# Autodesk Inventor assembly: dummy_pam_module_assembly
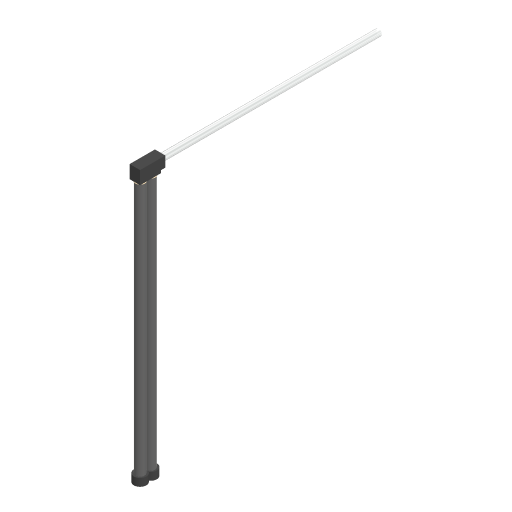
[picture p0: Inventor's stored thumbnail of the model, 512x512]
Saved by Autodesk Inventor 2024.3 (Build 283343000, 343)
## iProperties
Created: 2024-09-12
Part Number: dummy_pam_module_assembly
Document SubType Name: Assembly
Designer: gihyeok2
Author: gihyeok2
## Documents named in this file (10)
- C:\Users\gihyeok2\Desktop\New folder\component\mckibben_pam_module\dummy_pam_module_assembly.iam
- C:\Users\gihyeok2\Desktop\New folder\component\mckibben_pam_module\dummy_mckibben_pam_tube_4mm.ipt
- C:\Users\gihyeok2\Desktop\New folder\component\mckibben_pam_module\dummy_connecting_tube_3mm.ipt
- C:\Users\gihyeok2\Desktop\New folder\component\mckibben_pam_module\terminal_end_4.1mm_5.7mm.ipt
- C:\Users\gihyeok2\Desktop\New folder\component\mckibben_pam_module\input_connector_3.2mm_air_inlet.ipt
- C:\Users\gihyeok2\Desktop\New folder\component\mckibben_pam_module\dummy_air_tube_3mm.ipt
- C:\Users\gihyeok2\Desktop\New folder\component\mckibben_pam_module\dummy_sleeve_fixation_string.ipt
- C:\Users\gihyeok2\Desktop\New folder\component\mckibben_pam_module\input_connector_3.2mm_2ea.ipt
- C:\Users\gihyeok2\Desktop\New folder\component\mckibben_pam_module\dummy_terminal_wire_cut_3mm.ipt
- C:\Users\gihyeok2\Desktop\New folder\component\mckibben_pam_module\dummy_mckibben_pam_sleeve_4.2mm_cut.ipt
## Components (15 placed, 9 different names)
1. input_connector_3.2mm_2ea:1 — Mate:1, Flush:1, Mate:2, Mate:8, Mate:9, Mate:11, Mate:16, Mate:17, Mate:18, Mate:23, Mate:24
2. input_connector_3.2mm_air_inlet:1 — Mate:1, Flush:1, Mate:2, Mate:19, Mate:20
3. dummy_mckibben_pam_tube_4mm:1 — Mate:4, Flush:2, Mate:8, Mate:16, Mate:21, Flush:4, Flush:6
4. dummy_sleeve_fixation_string:1 — Mate:18
5. dummy_connecting_tube_3mm:1 — Mate:4, Flush:2
6. dummy_mckibben_pam_tube_4mm:2 — Mate:9, Mate:11, Mate:22, Flush:7
7. dummy_sleeve_fixation_string:2 — Mate:17
8. dummy_connecting_tube_3mm:2
9. dummy_air_tube_3mm:1 — Mate:19, Mate:20
10. terminal_end_4.1mm_5.7mm:1 — Mate:27, Flush:6
11. terminal_end_4.1mm_5.7mm:2 — Mate:28, Flush:7, Flush:8
12. dummy_terminal_wire_cut_3mm:1 — Mate:25, Flush:4
13. dummy_mckibben_pam_sleeve_4.2mm_cut:1 — Mate:21, Mate:23, Mate:25, Mate:27
14. dummy_mckibben_pam_sleeve_4.2mm_cut:2 — Mate:22, Mate:24, Mate:28, Mate:29
15. dummy_terminal_wire_cut_3mm:2 — Mate:29, Flush:8
## Relationships (27: Mate 20, Flush 7)
- Mate:1: input_connector_3.2mm_2ea:1 ↔ input_connector_3.2mm_air_inlet:1
- Flush:1: input_connector_3.2mm_2ea:1 ↔ input_connector_3.2mm_air_inlet:1
- Mate:2: input_connector_3.2mm_2ea:1 ↔ input_connector_3.2mm_air_inlet:1
- Mate:4: dummy_mckibben_pam_tube_4mm:1 ↔ dummy_connecting_tube_3mm:1
- Flush:2 (2 mm): dummy_mckibben_pam_tube_4mm:1 ↔ dummy_connecting_tube_3mm:1
- [Mate]: dummy_mckibben_pam_tube_4mm:2 ↔ dummy_connecting_tube_3mm:2
- [Flush] (2 mm): dummy_mckibben_pam_tube_4mm:2 ↔ dummy_connecting_tube_3mm:2
- Mate:8: input_connector_3.2mm_2ea:1 ↔ dummy_mckibben_pam_tube_4mm:1
- Mate:9: input_connector_3.2mm_2ea:1 ↔ dummy_mckibben_pam_tube_4mm:2
- Mate:11: input_connector_3.2mm_2ea:1 ↔ dummy_mckibben_pam_tube_4mm:2
- Mate:16: input_connector_3.2mm_2ea:1 ↔ dummy_mckibben_pam_tube_4mm:1
- Mate:17 (0.5 mm): input_connector_3.2mm_2ea:1 ↔ dummy_sleeve_fixation_string:2
- Mate:18 (0.5 mm): input_connector_3.2mm_2ea:1 ↔ dummy_sleeve_fixation_string:1
- Mate:19: input_connector_3.2mm_air_inlet:1 ↔ dummy_air_tube_3mm:1
- Mate:20: input_connector_3.2mm_air_inlet:1 ↔ dummy_air_tube_3mm:1
- Mate:21: dummy_mckibben_pam_tube_4mm:1 ↔ dummy_mckibben_pam_sleeve_4.2mm_cut:1
- Mate:22: dummy_mckibben_pam_tube_4mm:2 ↔ dummy_mckibben_pam_sleeve_4.2mm_cut:2
- Mate:23: input_connector_3.2mm_2ea:1 ↔ dummy_mckibben_pam_sleeve_4.2mm_cut:1
- Mate:24: input_connector_3.2mm_2ea:1 ↔ dummy_mckibben_pam_sleeve_4.2mm_cut:2
- Mate:25: dummy_terminal_wire_cut_3mm:1 ↔ dummy_mckibben_pam_sleeve_4.2mm_cut:1
- Flush:4: dummy_mckibben_pam_tube_4mm:1 ↔ dummy_terminal_wire_cut_3mm:1
- Mate:27: terminal_end_4.1mm_5.7mm:1 ↔ dummy_mckibben_pam_sleeve_4.2mm_cut:1
- Mate:28: terminal_end_4.1mm_5.7mm:2 ↔ dummy_mckibben_pam_sleeve_4.2mm_cut:2
- Flush:6: dummy_mckibben_pam_tube_4mm:1 ↔ terminal_end_4.1mm_5.7mm:1
- Flush:7: dummy_mckibben_pam_tube_4mm:2 ↔ terminal_end_4.1mm_5.7mm:2
- Mate:29: dummy_mckibben_pam_sleeve_4.2mm_cut:2 ↔ dummy_terminal_wire_cut_3mm:2
- Flush:8: terminal_end_4.1mm_5.7mm:2 ↔ dummy_terminal_wire_cut_3mm:2
## Named parameters: d90_d87 = 0 mm, d91_d88 = 2 mm
